# Autodesk Inventor assembly: body_struct
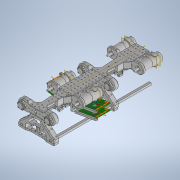
[picture p0: Inventor's stored thumbnail of the model, 180x180]
Saved by Autodesk Inventor 2020 (Build 240168000, 168)
## iProperties
Created: 2019-05-16
Part Number: body_struct
Document SubType Name: Assembly
Designer: psrob
Author: psrob
## Documents named in this file (18)
- E:\projects-2\project dog gen2\hardware\body_struct.iam
- E:\projects-2\project dog gen2\hardware\leg_ass_1.iam
- E:\projects-2\project dog gen2\hardware\carbon_fiber_200.ipt
- E:\projects-2\project dog gen2\hardware\body_bone_1.ipt
- E:\projects-2\project dog gen2\hardware\body_bone_2.ipt
- E:\projects-2\project dog gen2\hardware\body_bone_3.ipt
- E:\projects-2\project dog gen2\hardware\body_bone_4.ipt
- E:\projects-2\project dog gen2\hardware\body_bone_5.ipt
- E:\projects-2\project dog gen2\hardware\body_carbon_fiber_holder_1.ipt
- E:\projects-2\project dog gen2\hardware\pcb_holder_1.ipt
- E:\projects-2\project dog gen2\hardware\pcb_holder_2.ipt
- E:\projects-2\project dog gen2\hardware\motor_holder_1.ipt
- E:\projects-2\project dog gen2\hardware\switch_holder_5.ipt
- E:\projects-2\project dog gen2\hardware\ele_3d_3\dog_driver_5.brd.iam
- E:\projects-2\project dog gen2\hardware\pcb_shell_n1.ipt
- E:\projects-2\project dog gen2\hardware\pcb_shell_n1_MIR.ipt
- E:\projects-2\project dog gen2\hardware\carbon_fiber_fixer_1.ipt
- E:\projects-2\project dog gen2\hardware\leg_ass_1_MIR1.iam
## Components (33 placed, 17 different names)
1. leg_ass_1:1 [sub-assembly] — Flush:2, Flush:3, Flush:4, Insert:6, Flush:14, Insert:8, Insert:54
2. leg_ass_1:2 [sub-assembly] — Flush:2, Flush:3, Flush:4, Mate:1, Mate:2, Flush:5, Flush:10, Flush:12, Insert:1, Insert:4, Insert:10, Insert:11, Flush:27
3. carbon_fiber_200:1 — Mate:1, Mate:2, Flush:5
4. body_bone_1:1 — Flush:10, Insert:4, Insert:17, Insert:18, Insert:23, Insert:24, Insert:51
5. body_bone_2:1 — Insert:6, Insert:19, Insert:20, Insert:21, Insert:22, Insert:52
6. body_bone_3:1 — Flush:12, Insert:1, Insert:58
7. body_bone_4:1 — Insert:10, Insert:13, Insert:14, Insert:35, Insert:36, Insert:57
8. body_bone_5:1 — Flush:14, Insert:8, Mate:11, Flush:36, Insert:33, Insert:34, Insert:53, Insert:54, Insert:55, Insert:56
9. body_bone_1:2 — Insert:11, Insert:15, Insert:16, Flush:28, Insert:30, Angle:1, Insert:37, Insert:69
10. body_carbon_fiber_holder_1:1 — Flush:27, Insert:13, Insert:14, Mate:12, Flush:29, Mate:13, Flush:30, Mate:14, Mate:15, Flush:40
11. body_carbon_fiber_holder_1:2 — Insert:15, Insert:16, Insert:67, Insert:68
12. pcb_holder_1:1 — Flush:28, Insert:30, Flush:37, Insert:37, Mate:16, Flush:38, Insert:38, Insert:47, Insert:48, Insert:59, Insert:60, Insert:61, Insert:62
13. pcb_holder_2:1 — Mate:11, Insert:55, Insert:56
14. carbon_fiber_200:3 — Mate:13, Flush:30, Mate:14
15. carbon_fiber_200:4 — Mate:12, Flush:29, Mate:15
16. motor_holder_1:1 — Insert:17, Insert:18
17. motor_holder_1:2 — Insert:19, Insert:20, Insert:53
18. motor_holder_1:3 — Insert:23, Insert:24
19. motor_holder_1:4 — Insert:21, Insert:22
20. switch_holder_5:1 — Flush:36, Insert:33, Insert:34
21. switch_holder_5:2 — Insert:35, Insert:36
22. dog_driver_5.brd:1 [sub-assembly] — Flush:37, Angle:1, Mate:16, Flush:39, Mate:17
23. pcb_shell_n1:1 — Flush:38, Flush:39, Insert:38, Mate:17
24. dog_driver_5.brd:2 [sub-assembly] — Insert:63, Insert:64
25. dog_driver_5.brd:3 [sub-assembly] — Insert:65, Insert:66
26. pcb_shell_n1:2 — Insert:47, Insert:48, Insert:49, Insert:50
27. dog_driver_5.brd:4 [sub-assembly] — Insert:49, Insert:50
28. carbon_fiber_fixer_1:1 — Flush:40
29. leg_ass_1_MIR1:1 [sub-assembly] — Insert:51, Insert:52, Insert:69
30. pcb_shell_n1_MIR:3 — Insert:59, Insert:60, Insert:63, Insert:64
31. leg_ass_1_MIR1:2 [sub-assembly] — Insert:57, Insert:58
32. pcb_shell_n1_MIR:4 — Insert:61, Insert:62, Insert:65, Insert:66
33. carbon_fiber_fixer_1:2 — Insert:67, Insert:68
## Relationships (74: Insert 48, Flush 16, Mate 9, Angle 1)
- Flush:2: leg_ass_1:1 ↔ leg_ass_1:2
- Flush:3 (180 mm): leg_ass_1:1 ↔ leg_ass_1:2
- Flush:4: leg_ass_1:1 ↔ leg_ass_1:2
- Mate:1: leg_ass_1:2 ↔ carbon_fiber_200:1
- Mate:2: leg_ass_1:2 ↔ carbon_fiber_200:1
- Flush:5 (10 mm): leg_ass_1:2 ↔ carbon_fiber_200:1
- Flush:10: leg_ass_1:2 ↔ body_bone_1:1
- Flush:12: leg_ass_1:2 ↔ body_bone_3:1
- Insert:1: leg_ass_1:2 ↔ body_bone_3:1
- Insert:4: leg_ass_1:2 ↔ body_bone_1:1
- Insert:6: leg_ass_1:1 ↔ body_bone_2:1
- Flush:14: leg_ass_1:1 ↔ body_bone_5:1
- Insert:8: leg_ass_1:1 ↔ body_bone_5:1
- Insert:10: leg_ass_1:2 ↔ body_bone_4:1
- Insert:11: leg_ass_1:2 ↔ body_bone_1:2
- Flush:27: leg_ass_1:2 ↔ body_carbon_fiber_holder_1:1
- Insert:13: body_bone_4:1 ↔ body_carbon_fiber_holder_1:1
- Insert:14: body_bone_4:1 ↔ body_carbon_fiber_holder_1:1
- Insert:15: body_bone_1:2 ↔ body_carbon_fiber_holder_1:2
- Insert:16: body_bone_1:2 ↔ body_carbon_fiber_holder_1:2
- Flush:28: body_bone_1:2 ↔ pcb_holder_1:1
- Mate:11: body_bone_5:1 ↔ pcb_holder_2:1
- Mate:12: body_carbon_fiber_holder_1:1 ↔ carbon_fiber_200:4
- Flush:29: body_carbon_fiber_holder_1:1 ↔ carbon_fiber_200:4
- Mate:13: body_carbon_fiber_holder_1:1 ↔ carbon_fiber_200:3
- Flush:30: body_carbon_fiber_holder_1:1 ↔ carbon_fiber_200:3
- Mate:14: body_carbon_fiber_holder_1:1 ↔ carbon_fiber_200:3
- Mate:15: body_carbon_fiber_holder_1:1 ↔ carbon_fiber_200:4
- Insert:17: body_bone_1:1 ↔ motor_holder_1:1
- Insert:18: body_bone_1:1 ↔ motor_holder_1:1
- Insert:19: body_bone_2:1 ↔ motor_holder_1:2
- Insert:20: body_bone_2:1 ↔ motor_holder_1:2
- Insert:21: body_bone_2:1 ↔ motor_holder_1:4
- Insert:22: body_bone_2:1 ↔ motor_holder_1:4
- Insert:23: body_bone_1:1 ↔ motor_holder_1:3
- Insert:24: body_bone_1:1 ↔ motor_holder_1:3
- Insert:30: body_bone_1:2 ↔ pcb_holder_1:1
- Flush:36: body_bone_5:1 ↔ switch_holder_5:1
- Insert:33: body_bone_5:1 ↔ switch_holder_5:1
- Insert:34: body_bone_5:1 ↔ switch_holder_5:1
- Insert:35: body_bone_4:1 ↔ switch_holder_5:2
- Insert:36: body_bone_4:1 ↔ switch_holder_5:2
- Flush:37 (-5 mm): pcb_holder_1:1 ↔ dog_driver_5.brd:1
- Angle:1 (170 deg): body_bone_1:2 ↔ dog_driver_5.brd:1
- Insert:37: body_bone_1:2 ↔ pcb_holder_1:1
- Mate:16 (3 mm): pcb_holder_1:1 ↔ dog_driver_5.brd:1
- Flush:38: pcb_holder_1:1 ↔ pcb_shell_n1:1
- Flush:39: dog_driver_5.brd:1 ↔ pcb_shell_n1:1
- Insert:38: pcb_holder_1:1 ↔ pcb_shell_n1:1
- Insert:47: pcb_holder_1:1 ↔ pcb_shell_n1:2
- Insert:48: pcb_holder_1:1 ↔ pcb_shell_n1:2
- Insert:49: pcb_shell_n1:2 ↔ dog_driver_5.brd:4
- Insert:50: pcb_shell_n1:2 ↔ dog_driver_5.brd:4
- Flush:40: body_carbon_fiber_holder_1:1 ↔ carbon_fiber_fixer_1:1
- Insert:51: body_bone_1:1 ↔ leg_ass_1_MIR1:1
- Insert:52: body_bone_2:1 ↔ leg_ass_1_MIR1:1
- Insert:53: body_bone_5:1 ↔ motor_holder_1:2
- Insert:54: leg_ass_1:1 ↔ body_bone_5:1
- Insert:55: body_bone_5:1 ↔ pcb_holder_2:1
- Insert:56: body_bone_5:1 ↔ pcb_holder_2:1
- Insert:57: body_bone_4:1 ↔ leg_ass_1_MIR1:2
- Insert:58: body_bone_3:1 ↔ leg_ass_1_MIR1:2
- Insert:59: pcb_holder_1:1 ↔ pcb_shell_n1_MIR:3
- Insert:60: pcb_holder_1:1 ↔ pcb_shell_n1_MIR:3
- Insert:61: pcb_holder_1:1 ↔ pcb_shell_n1_MIR:4
- Insert:62: pcb_holder_1:1 ↔ pcb_shell_n1_MIR:4
- Insert:63: dog_driver_5.brd:2 ↔ pcb_shell_n1_MIR:3
- Insert:64: dog_driver_5.brd:2 ↔ pcb_shell_n1_MIR:3
- Insert:65: dog_driver_5.brd:3 ↔ pcb_shell_n1_MIR:4
- Insert:66: dog_driver_5.brd:3 ↔ pcb_shell_n1_MIR:4
- Insert:67: body_carbon_fiber_holder_1:2 ↔ carbon_fiber_fixer_1:2
- Insert:68: body_carbon_fiber_holder_1:2 ↔ carbon_fiber_fixer_1:2
- Insert:69: body_bone_1:2 ↔ leg_ass_1_MIR1:1
- Mate:17: dog_driver_5.brd:1 ↔ pcb_shell_n1:1
